# Autodesk Inventor assembly: TL20240701-10300SB-000
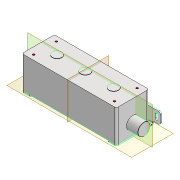
[picture p0: Inventor's stored thumbnail of the model, 180x180]
Saved by Autodesk Inventor 2022.5 (Build 265521000, 521)
## iProperties
Category: Title of a parent object over this object
Company: Customer
RuleStatus: InUse
Created: 2024-08-22
Part Number: TL20240701-10300SB-000
Project: Project Number
Checked By: Designed
Engr Approved By: Checked
User Status: set
Material: SS400
Description: Description
Document SubType Name: Assembly
Mfg Approved By: Approved
Designer: USER106
Stock Number: Stock Number
Deteil Description: Detail Description
Title: This Unit Title
Subject: Project Name
Author: USER106
Revision Number: A
## Documents named in this file (3)
- D:\V\Designs\프로젝트 자산\자동화 & 스마트팩토리\현대트랜시스(구 다이모스, 파워텍)\현대트랜시스(대유화성공장)_SW 시트조립라인\2.제작도면\1. 1ST LINE\SWITCH BOX\TL20240701-10200SB\TL20240701-10200SB-000.iam
- D:\V\Designs\프로젝트 자산\자동화 & 스마트팩토리\현대트랜시스(구 다이모스, 파워텍)\현대트랜시스(대유화성공장)_SW 시트조립라인\2.제작도면\기타(도면용 구성품)\구매품\TL20240701-3구 스위치 박스.ipt
- D:\V\Designs\프로젝트 자산\자동화 & 스마트팩토리\현대트랜시스(구 다이모스, 파워텍)\현대트랜시스(대유화성공장)_SW 시트조립라인\2.제작도면\1. 1ST LINE\SWITCH BOX\TL20240701-10200SB\TL20240701-10200SB-001.ipt
## Components (2 placed, 2 different names)
1. TL20240701-10200SB-001:1 — Flush:1, Flush:2, Flush:3, Mate:1, Mate:2, Mate:3
2. TL20240701-3구 스위치 박스:1 — Mate:1, Mate:2, Mate:3
## Relationships (6: Flush 3, Mate 3)
- Flush:1: TL20240701-10200SB-001:1
- Flush:2: TL20240701-10200SB-001:1
- Flush:3: TL20240701-10200SB-001:1
- Mate:1: TL20240701-10200SB-001:1 ↔ TL20240701-3구 스위치 박스:1
- Mate:2: TL20240701-10200SB-001:1 ↔ TL20240701-3구 스위치 박스:1
- Mate:3: TL20240701-10200SB-001:1 ↔ TL20240701-3구 스위치 박스:1
